# Autodesk Inventor assembly: Assembly2
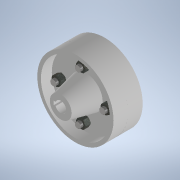
[picture p0: Inventor's stored thumbnail of the model, 180x180]
Saved by Autodesk Inventor 2021 (Build 250183000, 183)
## iProperties
Created: 2021-05-13
Part Number: Assembly2
Document SubType Name: Assembly
Designer: peris
Author: peris
## Documents named in this file (5)
- D:\Inventor\nm20003_Assembly2.iam
- D:\Inventor\nm20003_Part2.1.ipt
- C:\Users\peris\OneDrive\Έγγραφα\Inventor\Content Center Files\R2021\en-US\ISO 4017(1)\ISO 4017 - M16 x 45 - ISO.ipt
- D:\Inventor\nm20003_Part2.2.ipt
- C:\Users\peris\OneDrive\Έγγραφα\Inventor\Content Center Files\R2021\en-US\ISO 4033(2)\ISO 4033 - M16 - ISO.ipt
## Components (10 placed, 4 different names)
1. nm20003_Part2.1:1 — Cylindrical:1, Symmetry:1, Insert:2, Flush:1
2. nm20003_Part2.2:1 — Cylindrical:1, Symmetry:1, Insert:1, Flush:1
3. ISO 4017 M16 x 45:1 — Insert:1
4. ISO 4033 M16:1 — Insert:2
5. ISO 4017 M16 x 45:2
6. ISO 4033 M16:2
7. ISO 4017 M16 x 45:3
8. ISO 4033 M16:3
9. ISO 4017 M16 x 45:4
10. ISO 4033 M16:4
## Component patterns: (4 elements, first: ISO 4017 M16 x 45:1 + ISO 4033 M16:1)
## Relationships (5: Insert 2, CylindricalJoint 1, Symmetry 1, Flush 1)
- Cylindrical:1: nm20003_Part2.1:1 ↔ nm20003_Part2.2:1
- Symmetry:1: nm20003_Part2.1:1 ↔ nm20003_Part2.2:1
- Insert:1: nm20003_Part2.2:1 ↔ ISO 4017 M16 x 45:1
- Insert:2: nm20003_Part2.1:1 ↔ ISO 4033 M16:1
- Flush:1: nm20003_Part2.1:1 ↔ nm20003_Part2.2:1
